# Autodesk Inventor assembly: HbHand_MIR1
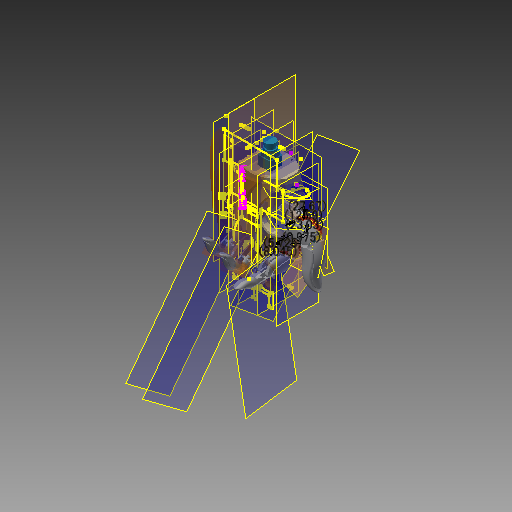
[picture p0: Inventor's stored thumbnail of the model, 512x512]
Saved by Autodesk Inventor 2017.3 (Build 213256000, 256)
## iProperties
Part Number: HbHand_MIR1
Material: 一般
Document SubType Name: Assembly
Designer: sktom
Author: sktom
## Documents named in this file (21)
- D:\CloudStrage\OneDrive\CAD\MAJ\hackberry\HACKberry-hardware\3D_69%inlength\Inventor\HbHandForChild\HbHand_MIR1.iam
- D:\CloudStrage\OneDrive\CAD\MAJ\hackberry\HACKberry-hardware\3D_69%inlength\Inventor\HbHandForChild\HbPalmBase03ForChild_MIR1.ipt
- D:\CloudStrage\OneDrive\CAD\MAJ\hackberry\HACKberry-hardware\3D_69%inlength\Inventor\HbHandForChild\bearing_683_MIR1.ipt
- D:\CloudStrage\OneDrive\CAD\MAJ\hackberry\HACKberry-hardware\3D_69%inlength\Inventor\HbHandForChild\HbthumbU02ForChild\HbthumbU02ForChild_MIR1.iam
- D:\CloudStrage\OneDrive\CAD\MAJ\hackberry\HACKberry-hardware\3D_69%inlength\Inventor\HbHandForChild\HbServoHK282A\Servo_HK282A_Hone_MIR1.ipt
- D:\CloudStrage\OneDrive\CAD\MAJ\hackberry\HACKberry-hardware\3D_69%inlength\Inventor\HbHandForChild\HbIndexFinger01ForChild\HbIndexFinger01ForChild_MIR1.iam
- D:\CloudStrage\OneDrive\CAD\MAJ\hackberry\HACKberry-hardware\3D_69%inlength\Inventor\HbHandForChild\HbFinger01ForChild\HbFinger01ForChild_MIR1.iam
- D:\CloudStrage\OneDrive\CAD\MAJ\hackberry\HACKberry-hardware\3D_69%inlength\Inventor\HbHandForChild\HbRing-LittleCouplerLink01ForChild_MIR1.ipt
- D:\CloudStrage\OneDrive\CAD\MAJ\hackberry\HACKberry-hardware\3D_69%inlength\Inventor\HbHandForChild\HbMiddle-RingCouplerLink01ForChild_MIR1.ipt
- D:\CloudStrage\OneDrive\CAD\MAJ\hackberry\HACKberry-hardware\3D_69%inlength\Inventor\HbHandForChild\servo\Tower Pro 9g Micro Servo SG90_MIR1.iam
- D:\CloudStrage\OneDrive\CAD\MAJ\hackberry\HACKberry-hardware\3D_69%inlength\Inventor\HbHandForChild\DummyASV-15MG_MIR1.ipt
- D:\CloudStrage\OneDrive\CAD\MAJ\hackberry\HACKberry-hardware\3D_69%inlength\Inventor\HbHandForChild\HbWristMount01ForChild_MIR1.ipt
- D:\CloudStrage\OneDrive\CAD\MAJ\hackberry\HACKberry-hardware\3D_69%inlength\Inventor\HbHandForChild\HbFingerMainCouplerLink01ForChild_MIR1.ipt
- D:\CloudStrage\OneDrive\CAD\MAJ\hackberry\HACKberry-hardware\3D_69%inlength\Inventor\HbHandForChild\DummyASV-15MGSingleHorn01_MIR1.ipt
- D:\CloudStrage\OneDrive\CAD\MAJ\hackberry\HACKberry-hardware\3D_69%inlength\Inventor\HbHandForChild\HbBackCover02ForChild_MIR1.ipt
- D:\CloudStrage\OneDrive\CAD\MAJ\hackberry\HACKberry-hardware\3D_69%inlength\Inventor\HbHandForChild\Spur Gear (16 teeth)_MIR.ipt
- D:\CloudStrage\OneDrive\CAD\MAJ\hackberry\HACKberry-hardware\3D_69%inlength\Inventor\HbHandForChild\spacer_2_3_l3.5_MIR.ipt
- D:\CloudStrage\OneDrive\CAD\MAJ\hackberry\HACKberry-hardware\3D_69%inlength\Inventor\HbHandForChild\HbServoCover_MIR.ipt
- D:\CloudStrage\OneDrive\CAD\MAJ\hackberry\HACKberry-hardware\3D_69%inlength\Inventor\HbHandForChild\HbShaftStopperB04ForChild_MIR.ipt
- D:\CloudStrage\OneDrive\CAD\MAJ\hackberry\HACKberry-hardware\3D_69%inlength\Inventor\HbHandForChild\HbShaftStopperA04ForChild_MIR.ipt
- D:\CloudStrage\OneDrive\CAD\MAJ\hackberry\HACKberry-hardware\3D_69%inlength\Inventor\HbHandForChild\shaft_phi1.5_l10_MIR.ipt
## Components (33 placed, 20 different names)
1. HbPalmBase03ForChild_MIR1:1 — 挿入:1, 挿入:5, 挿入:4, 挿入:6, 挿入:8, 挿入:7, 挿入:10, 挿入:9, 挿入:12, 挿入:11, 挿入:16, 挿入:15, メイト:3, メイト:2, 挿入:18, 挿入:17, 挿入:23, 挿入:22, 挿入:32, 挿入:31, 挿入:34, 挿入:33, 挿入:35, 挿入:36, 挿入:37, 挿入:38, 挿入:39, 挿入:41, 挿入:40
2. bearing_683_MIR1:1 — 挿入:1, 挿入:2
3. HbthumbU02ForChild_MIR1:1 [sub-assembly] — 挿入:2, 挿入:3
4. Servo_HK282A_Hone_MIR1:1 — 挿入:5, 挿入:4, 挿入:3
5. HbIndexFinger01ForChild_MIR1:1 [sub-assembly] — 挿入:6
6. HbFinger01ForChild_MIR1:1 [sub-assembly] — 挿入:8, 挿入:7, 挿入:13, 挿入:30
7. HbFinger01ForChild_MIR1:2 [sub-assembly] — 挿入:10, 挿入:9, 挿入:14, 挿入:28, 挿入:29, 円柱状:1
8. HbFinger01ForChild_MIR1:3 [sub-assembly] — 挿入:12, 挿入:11, 挿入:19, 挿入:26, 挿入:27, 円柱状:2
9. HbRing-LittleCouplerLink01ForChild_MIR1:1 — 挿入:14, 円柱状:2
10. HbMiddle-RingCouplerLink01ForChild_MIR1:1 — 挿入:13, 円柱状:1
11. Tower Pro 9g Micro Servo SG90_MIR1:1 [sub-assembly] — 挿入:16, 挿入:15, 挿入:24
12. DummyASV-15MG_MIR1:1 — メイト:3, メイト:2, 挿入:20
13. HbWristMount01ForChild_MIR1:1 — 挿入:18, 挿入:17
14. HbFingerMainCouplerLink01ForChild_MIR1:1 — 挿入:19, 挿入:21
15. DummyASV-15MGSingleHorn01_MIR1:1 — 挿入:21, 挿入:20, 挿入:25
16. HbBackCover02ForChild_MIR1:1 — 挿入:23, 挿入:22
17. Spur Gear (16 teeth)_MIR:1 — 挿入:24
18. spacer_2_3_l3.5_MIR:1 — 挿入:26
19. spacer_2_3_l3.5_MIR:2 — 挿入:25
20. spacer_2_3_l3.5_MIR:3 — 挿入:27
21. spacer_2_3_l3.5_MIR:4 — 挿入:28
22. spacer_2_3_l3.5_MIR:5 — 挿入:29
23. spacer_2_3_l3.5_MIR:6 — 挿入:30
24. HbServoCover_MIR:1 — 挿入:32, 挿入:31
25. HbShaftStopperB04ForChild_MIR:1 — 挿入:34
26. HbShaftStopperA04ForChild_MIR:1 — 挿入:33
27. shaft_phi1.5_l10_MIR:1 — 挿入:35
28. shaft_phi1.5_l10_MIR:2 — 挿入:36
29. shaft_phi1.5_l10_MIR:3 — 挿入:37
30. shaft_phi1.5_l10_MIR:4 — 挿入:38
31. shaft_phi1.5_l10_MIR:5 — 挿入:39
32. shaft_phi1.5_l10_MIR:6 — 挿入:41
33. shaft_phi1.5_l10_MIR:7 — 挿入:40
## Relationships (45: Insert 41, Mate 2, CylindricalJoint 2)
- 挿入:1 [Insert]: HbPalmBase03ForChild_MIR1:1 ↔ bearing_683_MIR1:1
- 挿入:2 [Insert]: bearing_683_MIR1:1 ↔ HbthumbU02ForChild_MIR1:1
- 挿入:5 [Insert]: HbPalmBase03ForChild_MIR1:1 ↔ Servo_HK282A_Hone_MIR1:1
- 挿入:4 [Insert]: HbPalmBase03ForChild_MIR1:1 ↔ Servo_HK282A_Hone_MIR1:1
- 挿入:3 [Insert]: HbthumbU02ForChild_MIR1:1 ↔ Servo_HK282A_Hone_MIR1:1
- 挿入:6 [Insert]: HbPalmBase03ForChild_MIR1:1 ↔ HbIndexFinger01ForChild_MIR1:1
- 挿入:8 [Insert]: HbPalmBase03ForChild_MIR1:1 ↔ HbFinger01ForChild_MIR1:1
- 挿入:7 [Insert]: HbPalmBase03ForChild_MIR1:1 ↔ HbFinger01ForChild_MIR1:1
- 挿入:10 [Insert]: HbPalmBase03ForChild_MIR1:1 ↔ HbFinger01ForChild_MIR1:2
- 挿入:9 [Insert]: HbPalmBase03ForChild_MIR1:1 ↔ HbFinger01ForChild_MIR1:2
- 挿入:12 [Insert]: HbPalmBase03ForChild_MIR1:1 ↔ HbFinger01ForChild_MIR1:3
- 挿入:11 [Insert]: HbPalmBase03ForChild_MIR1:1 ↔ HbFinger01ForChild_MIR1:3
- 挿入:14 [Insert]: HbFinger01ForChild_MIR1:2 ↔ HbRing-LittleCouplerLink01ForChild_MIR1:1
- 挿入:13 [Insert]: HbFinger01ForChild_MIR1:1 ↔ HbMiddle-RingCouplerLink01ForChild_MIR1:1
- 挿入:16 [Insert]: HbPalmBase03ForChild_MIR1:1 ↔ Tower Pro 9g Micro Servo SG90_MIR1:1
- 挿入:15 [Insert]: HbPalmBase03ForChild_MIR1:1 ↔ Tower Pro 9g Micro Servo SG90_MIR1:1
- メイト:3 [Mate]: HbPalmBase03ForChild_MIR1:1 ↔ DummyASV-15MG_MIR1:1
- メイト:2 [Mate]: HbPalmBase03ForChild_MIR1:1 ↔ DummyASV-15MG_MIR1:1
- 挿入:18 [Insert]: HbPalmBase03ForChild_MIR1:1 ↔ HbWristMount01ForChild_MIR1:1
- 挿入:17 [Insert]: HbPalmBase03ForChild_MIR1:1 ↔ HbWristMount01ForChild_MIR1:1
- 挿入:19 [Insert] (0.1 mm): HbFinger01ForChild_MIR1:3 ↔ HbFingerMainCouplerLink01ForChild_MIR1:1
- 挿入:21 [Insert]: HbFingerMainCouplerLink01ForChild_MIR1:1 ↔ DummyASV-15MGSingleHorn01_MIR1:1
- 挿入:20 [Insert]: DummyASV-15MG_MIR1:1 ↔ DummyASV-15MGSingleHorn01_MIR1:1
- 挿入:23 [Insert]: HbPalmBase03ForChild_MIR1:1 ↔ HbBackCover02ForChild_MIR1:1
- 挿入:22 [Insert]: HbPalmBase03ForChild_MIR1:1 ↔ HbBackCover02ForChild_MIR1:1
- 挿入:24 [Insert] (0.8 mm): Tower Pro 9g Micro Servo SG90_MIR1:1 ↔ Spur Gear (16 teeth)_MIR:1
- 挿入:26 [Insert]: HbFinger01ForChild_MIR1:3 ↔ spacer_2_3_l3.5_MIR:1
- 挿入:25 [Insert]: DummyASV-15MGSingleHorn01_MIR1:1 ↔ spacer_2_3_l3.5_MIR:2
- 挿入:27 [Insert]: HbFinger01ForChild_MIR1:3 ↔ spacer_2_3_l3.5_MIR:3
- 挿入:28 [Insert]: HbFinger01ForChild_MIR1:2 ↔ spacer_2_3_l3.5_MIR:4
- 挿入:29 [Insert]: HbFinger01ForChild_MIR1:2 ↔ spacer_2_3_l3.5_MIR:5
- 挿入:30 [Insert]: HbFinger01ForChild_MIR1:1 ↔ spacer_2_3_l3.5_MIR:6
- 挿入:32 [Insert]: HbPalmBase03ForChild_MIR1:1 ↔ HbServoCover_MIR:1
- 挿入:31 [Insert]: HbPalmBase03ForChild_MIR1:1 ↔ HbServoCover_MIR:1
- 挿入:34 [Insert]: HbPalmBase03ForChild_MIR1:1 ↔ HbShaftStopperB04ForChild_MIR:1
- 挿入:33 [Insert]: HbPalmBase03ForChild_MIR1:1 ↔ HbShaftStopperA04ForChild_MIR:1
- 挿入:35 [Insert]: HbPalmBase03ForChild_MIR1:1 ↔ shaft_phi1.5_l10_MIR:1
- 挿入:36 [Insert] (0.5 mm): HbPalmBase03ForChild_MIR1:1 ↔ shaft_phi1.5_l10_MIR:2
- 挿入:37 [Insert] (0.3 mm): HbPalmBase03ForChild_MIR1:1 ↔ shaft_phi1.5_l10_MIR:3
- 挿入:38 [Insert] (0.3 mm): HbPalmBase03ForChild_MIR1:1 ↔ shaft_phi1.5_l10_MIR:4
- 挿入:39 [Insert] (0.5 mm): HbPalmBase03ForChild_MIR1:1 ↔ shaft_phi1.5_l10_MIR:5
- 挿入:41 [Insert] (0.5 mm): HbPalmBase03ForChild_MIR1:1 ↔ shaft_phi1.5_l10_MIR:6
- 挿入:40 [Insert] (0.5 mm): HbPalmBase03ForChild_MIR1:1 ↔ shaft_phi1.5_l10_MIR:7
- 円柱状:2 [CylindricalJoint]: HbFinger01ForChild_MIR1:3 ↔ HbRing-LittleCouplerLink01ForChild_MIR1:1
- 円柱状:1 [CylindricalJoint]: HbFinger01ForChild_MIR1:2 ↔ HbMiddle-RingCouplerLink01ForChild_MIR1:1
